# Autodesk Inventor assembly: Assieme prova
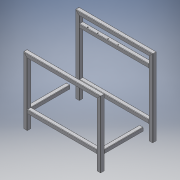
[picture p0: Inventor's stored thumbnail of the model, 180x180]
Saved by Autodesk Inventor 2018 (Build 220112000, 112)
## iProperties
Created: 2020-05-28
Part Number: Assieme prova
Material: Generico
Document SubType Name: Assembly
Designer: Francesco
Author: Francesco
## Documents named in this file (7)
- C:\Users\Francesco\Desktop\Prova Inventor\Assieme tubolari.iam
- C:\Users\Francesco\Desktop\Prova Inventor\Piantone tubolare l magg.ipt
- C:\Users\Francesco\Desktop\Prova Inventor\Tubolari horizontal.ipt
- C:\Users\Francesco\Desktop\Prova Inventor\Tubolari horizontal 45.ipt
- C:\Users\Francesco\Desktop\Prova Inventor\Tubolare horizontal corto.ipt
- C:\Users\Francesco\Desktop\Prova Inventor\Piantone tubolare l min.ipt
- C:\Users\Francesco\Desktop\Prova Inventor\Tubolari horizontal superiore.ipt
## Components (11 placed, 5 different names)
1. Piantone tubolare l magg:2 — Coincidente:2, Allineato:4, Coincidente:3, Allineato:7, Coincidente:4, Coincidente:13, Allineato:13
2. Piantone tubolare l magg:3 — Coincidente:7, Allineato:9, Coincidente:8, Coincidente:11, Allineato:11, Allineato:17, Coincidente:20, Allineato:22
3. Tubolari horizontal:1 — Allineato:3, Coincidente:19, Allineato:19, Allineato:20
4. Tubolari horizontal:2 — Allineato:3, Coincidente:2, Allineato:4, Allineato:12, Allineato:14
5. Tubolari horizontal 45:1 — Coincidente:3, Allineato:7, Coincidente:4, Coincidente:7, Allineato:9, Coincidente:8, Coincidente:21
6. Tubolari horizontal 45:2 — Coincidente:14, Allineato:15, Coincidente:15, Coincidente:16, Allineato:16, Coincidente:17
7. Tubolare horizontal corto:1 — Coincidente:11, Allineato:11, Allineato:12, Allineato:18, Coincidente:18, Allineato:21
8. Tubolare horizontal corto:2 — Coincidente:13, Allineato:13, Allineato:14, Allineato:20
9. Piantone tubolare l min:1 — Coincidente:14, Allineato:15, Coincidente:15, Coincidente:19, Allineato:19
10. Piantone tubolare l min:2 — Coincidente:16, Allineato:16, Coincidente:17, Allineato:17, Allineato:18, Coincidente:18, Allineato:21
11. Tubolari horizontal:3 — Coincidente:20, Allineato:22, Coincidente:21
## Relationships (31: Flush 16, Mate 15)
- Allineato:3 [Flush]: Tubolari horizontal:1 ↔ Tubolari horizontal:2
- Coincidente:2 [Mate]: Piantone tubolare l magg:2 ↔ Tubolari horizontal:2
- Allineato:4 [Flush]: Piantone tubolare l magg:2 ↔ Tubolari horizontal:2
- Coincidente:3 [Mate]: Piantone tubolare l magg:2 ↔ Tubolari horizontal 45:1
- Allineato:7 [Flush]: Piantone tubolare l magg:2 ↔ Tubolari horizontal 45:1
- Coincidente:4 [Mate]: Piantone tubolare l magg:2 ↔ Tubolari horizontal 45:1
- Coincidente:7 [Mate]: Piantone tubolare l magg:3 ↔ Tubolari horizontal 45:1
- Allineato:9 [Flush]: Piantone tubolare l magg:3 ↔ Tubolari horizontal 45:1
- Coincidente:8 [Mate]: Piantone tubolare l magg:3 ↔ Tubolari horizontal 45:1
- Coincidente:11 [Mate]: Piantone tubolare l magg:3 ↔ Tubolare horizontal corto:1
- Allineato:11 [Flush]: Piantone tubolare l magg:3 ↔ Tubolare horizontal corto:1
- Allineato:12 [Flush]: Tubolari horizontal:2 ↔ Tubolare horizontal corto:1
- Coincidente:13 [Mate]: Piantone tubolare l magg:2 ↔ Tubolare horizontal corto:2
- Allineato:13 [Flush]: Piantone tubolare l magg:2 ↔ Tubolare horizontal corto:2
- Allineato:14 [Flush]: Tubolari horizontal:2 ↔ Tubolare horizontal corto:2
- Coincidente:14 [Mate]: Tubolari horizontal 45:2 ↔ Piantone tubolare l min:1
- Allineato:15 [Flush]: Tubolari horizontal 45:2 ↔ Piantone tubolare l min:1
- Coincidente:15 [Mate]: Tubolari horizontal 45:2 ↔ Piantone tubolare l min:1
- Coincidente:16 [Mate]: Tubolari horizontal 45:2 ↔ Piantone tubolare l min:2
- Allineato:16 [Flush]: Tubolari horizontal 45:2 ↔ Piantone tubolare l min:2
- Coincidente:17 [Mate]: Tubolari horizontal 45:2 ↔ Piantone tubolare l min:2
- Allineato:17 [Flush]: Piantone tubolare l magg:3 ↔ Piantone tubolare l min:2
- Allineato:18 [Flush]: Tubolare horizontal corto:1 ↔ Piantone tubolare l min:2
- Coincidente:18 [Mate]: Tubolare horizontal corto:1 ↔ Piantone tubolare l min:2
- Coincidente:19 [Mate]: Tubolari horizontal:1 ↔ Piantone tubolare l min:1
- Allineato:19 [Flush]: Tubolari horizontal:1 ↔ Piantone tubolare l min:1
- Allineato:20 [Flush]: Tubolari horizontal:1 ↔ Tubolare horizontal corto:2
- Allineato:21 [Flush] (150 mm): Tubolare horizontal corto:1 ↔ Piantone tubolare l min:2
- Coincidente:20 [Mate]: Piantone tubolare l magg:3 ↔ Tubolari horizontal:3
- Allineato:22 [Flush]: Piantone tubolare l magg:3 ↔ Tubolari horizontal:3
- Coincidente:21 [Mate] (70 mm): Tubolari horizontal 45:1 ↔ Tubolari horizontal:3
